# Autodesk Inventor assembly: taiko
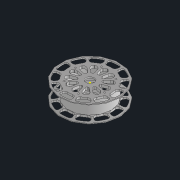
[picture p0: Inventor's stored thumbnail of the model, 180x180]
Saved by Autodesk Inventor 2022 (Build 260153000, 153)
## iProperties
Created: 2024-06-02
Part Number: taiko
Document SubType Name: Assembly
Designer: gisen
Author: gisen
## Documents named in this file (3)
- C:\Users\gisen\Documents\CAD\inventor\git\fishing\taiko.iam
- C:\Users\gisen\Documents\CAD\inventor\git\fishing\A6063-PP-65-2-30.ipt
- C:\Users\gisen\Documents\CAD\inventor\git\fishing\taiko_01.ipt
## Components (3 placed, 2 different names)
1. A6063-PP-65-2-30:1 — メイト:1, メイト:2, メイト:3, メイト:4
2. taiko_01:1 — メイト:1, メイト:2, メイト:5
3. taiko_01:2 — メイト:3, メイト:4, メイト:5
## Relationships (5: Mate 5)
- メイト:1 [Mate]: A6063-PP-65-2-30:1 ↔ taiko_01:1
- メイト:2 [Mate]: A6063-PP-65-2-30:1 ↔ taiko_01:1
- メイト:3 [Mate]: A6063-PP-65-2-30:1 ↔ taiko_01:2
- メイト:4 [Mate]: A6063-PP-65-2-30:1 ↔ taiko_01:2
- メイト:5 [Mate]: taiko_01:1 ↔ taiko_01:2
